# Autodesk Inventor assembly: PS20027
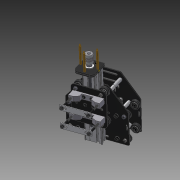
[picture p0: Inventor's stored thumbnail of the model, 180x180]
Saved by Autodesk Inventor 2014 (Build 180170000, 170)
## iProperties
Created: 2013-03-06
Part Number: PS20027
Document SubType Name: Assembly
Designer: Edward
Mass: 1567.3 g
Surface Area: 2632.04 cm^2
Volume: 388.503 cm^3
Density: 4.03421 g/cm^3
Author: Edward
## Documents named in this file (34)
- C:\Users\Edward\Documents\GitHub\Shapeoko_2\Autodesk_Inventor_Project\PS20027.iam
- C:\Users\Edward\Documents\GitHub\Shapeoko_2\Autodesk_Inventor_Project\25142-07.ipt
- C:\Users\Edward\Documents\GitHub\Shapeoko_2\Autodesk_Inventor_Project\25287-02.ipt
- C:\Users\Edward\Documents\GitHub\Shapeoko_2\Autodesk_Inventor_Project\25284-02.ipt
- C:\Users\Edward\Documents\GitHub\Shapeoko_2\Autodesk_Inventor_Project\25287-03.ipt
- C:\Users\Edward\Documents\GitHub\Shapeoko_2\Autodesk_Inventor_Project\PS20021.iam
- C:\Users\Edward\Documents\GitHub\Shapeoko_2\Autodesk_Inventor_Project\26016-01.ipt
- C:\Users\Edward\Documents\GitHub\Shapeoko_2\Autodesk_Inventor_Project\PS20002.ipt
- C:\Users\Edward\Documents\GitHub\Shapeoko_2\Autodesk_Inventor_Project\PS20005.ipt
- C:\Users\Edward\Documents\GitHub\Shapeoko_2\Autodesk_Inventor_Project\PS20014.ipt
- C:\Users\Edward\Documents\GitHub\Shapeoko_2\Autodesk_Inventor_Project\25286-01.ipt
- C:\Users\Edward\Documents\GitHub\Shapeoko_2\Autodesk_Inventor_Project\25772-02.ipt
- C:\Users\Edward\Documents\GitHub\Shapeoko_2\Autodesk_Inventor_Project\PS20011.ipt
- C:\Users\Edward\Documents\GitHub\Shapeoko_2\Autodesk_Inventor_Project\PS20007.ipt
- C:\Users\Edward\Documents\GitHub\Shapeoko_2\Autodesk_Inventor_Project\30288-01.ipt
- C:\Users\Edward\Documents\GitHub\Shapeoko_2\Autodesk_Inventor_Project\30169-01.ipt
- C:\Users\Edward\Documents\GitHub\Shapeoko_2\Autodesk_Inventor_Project\30289-01.ipt
- C:\Users\Edward\Documents\GitHub\Shapeoko_2\Autodesk_Inventor_Project\30287-01.ipt
- C:\Users\Edward\Documents\GitHub\Shapeoko_2\Autodesk_Inventor_Project\PS20015.ipt
- C:\Users\Edward\Documents\GitHub\Shapeoko_2\Autodesk_Inventor_Project\25286-02.ipt
- C:\Users\Edward\Documents\GitHub\Shapeoko_2\Autodesk_Inventor_Project\PS20010.ipt
- C:\Users\Edward\Documents\GitHub\Shapeoko_2\Autodesk_Inventor_Project\30158-01.ipt
- C:\Users\Edward\Documents\GitHub\Shapeoko_2\Autodesk_Inventor_Project\25203-02.iam
- C:\Users\Edward\Documents\GitHub\Shapeoko_2\Autodesk_Inventor_Project\25312-14.ipt
- C:\Users\Edward\Documents\GitHub\Shapeoko_2\Autodesk_Inventor_Project\25286-05.ipt
- C:\Users\Edward\Documents\GitHub\Shapeoko_2\Autodesk_Inventor_Project\PS20012.ipt
- C:\Users\Edward\Documents\GitHub\Shapeoko_2\Autodesk_Inventor_Project\PS20013.ipt
- C:\Users\Edward\Documents\GitHub\Shapeoko_2\Autodesk_Inventor_Project\25285-10.ipt
- C:\Users\Edward\Documents\GitHub\Shapeoko_2\Autodesk_Inventor_Project\PS20016.ipt
- C:\Users\Edward\Documents\GitHub\Shapeoko_2\Autodesk_Inventor_Project\PS20022.iam
- C:\Users\Edward\Documents\GitHub\Shapeoko_2\Autodesk_Inventor_Project\25312-20.ipt
- C:\Users\Edward\Documents\GitHub\Shapeoko_2\Autodesk_Inventor_Project\PS20006.ipt
- C:\Users\Edward\Documents\GitHub\Shapeoko_2\Autodesk_Inventor_Project\PS20004.ipt
- C:\Users\Edward\Documents\GitHub\Shapeoko_2\Autodesk_Inventor_Project\PS20017.ipt
## Components (147 placed, 34 different names)
1. 25142-07:1 — Mate:10, Flush:11, Flush:15, Mate:23, Mate:24, Flush:17, Insert:128, Insert:129, Angle:2, Mate:49, Flush:25
2. PS20021:1 [sub-assembly] — Mate:10, Flush:11, Flush:15, Flush:16, Insert:218, Insert:220, Insert:233, Insert:235, Insert:238, Insert:239, Insert:241, Insert:243, Insert:245, Insert:247, Insert:249, Insert:251
3. 25772-02:1
4. 30288-01:1 — Mate:25, Mate:26, Mate:28, Flush:17, Insert:115, Insert:116, Insert:117, Mate:32, Flush:18, Mate:47, Mate:48
5. 30288-01:2 — Insert:108, Mate:28, Insert:131, Insert:132, Insert:133
6. 30169-01:1 — Insert:108, Mate:25, Mate:26, Insert:109, Insert:110, Mate:53
7. PS20007:1 — Insert:109
8. PS20007:2 — Insert:110
9. 25287-03:2 — Insert:115, Insert:188
10. 25287-03:3 — Insert:116, Insert:187
11. 25287-03:4 — Insert:117, Insert:186
12. 30289-01:1 — Insert:128, Insert:129, Mate:32, Insert:136, Insert:137, Flush:18
13. PS20011:2 — Mate:33
14. 30287-01:1 — Insert:140, Insert:141, Insert:152, Angle:2, Mate:37, Insert:153, Insert:156, Insert:158, Insert:159, Insert:160, Insert:161, Insert:165, Insert:166, Mate:39, Insert:172, Mate:42, Insert:181, Insert:194, Insert:195, Mate:49, Flush:25
15. PSM3-01 — Insert:133, Insert:191
16. PS20015:4 — Insert:132, Insert:192
17. PS20015:5 — Insert:131, Insert:193
18. PS20004:9 — Insert:134
19. 25287-02:36 — Insert:134, Insert:136
20. PS20004:8 — Insert:135
21. 25287-02:37 — Insert:135, Insert:137
22. PS20010:1 — Insert:140, Insert:141, Mate:33
23. 30158-01:4 — Insert:152, Mate:38
24. 25287-02:45 — Insert:156, Insert:157
25. 25203-02:7 [sub-assembly] — Mate:37, Insert:154, Insert:155
26. 25284-02:13 — Insert:157
27. 25312-14:1 — Insert:153, Insert:154
28. 25286-05:1 — Insert:155
29. PS20012:1 — Insert:158, Insert:159, Insert:179, Mate:50, Flush:26, Flush:27, Insert:197
30. PS20012:2 — Insert:160, Insert:161, Mate:51, Flush:28, Flush:29, Mate:52
31. 25287-02:48 — Insert:166
32. 25203-02:8 [sub-assembly]
33. 25284-02:15
34. 25312-14:2 — Insert:165
35. 25286-05:2
36. 25203-02:9 [sub-assembly]
37. 25312-14:3 — Mate:38, Mate:39
38. 25286-05:3
39. 30158-01:5 — Insert:172, Mate:41
40. 25203-02:10 [sub-assembly]
41. 25312-14:4 — Mate:41, Mate:42
42. 25286-05:4
43. PS20016:1 — Mate:47, Insert:189
44. PS20016:2 — Mate:48, Insert:190
45. PS20014:9
46. PS20014:11
47. PS20014:12
48. 25285-10:1 — Insert:188
49. 25285-10:2 — Insert:187
50. 25285-10:3 — Insert:186
51. PS20016:3 — Insert:189
52. PS20016:4 — Insert:190
53. PS20015:6 — Insert:191
54. PS20015:7 — Insert:192
55. PS20015:8 — Insert:193
56. 25286-02:10 — Insert:194
57. 25286-02:11 — Insert:195
58. PS20013:3 — Mate:50, Flush:26, Flush:27, Mate:51
59. PS20013:4 — Flush:28, Flush:29, Mate:52
60. PS20022:1 [sub-assembly] — Insert:201, Insert:204, Insert:207, Insert:210, Insert:212, Insert:214, Insert:215, Insert:216, Insert:221, Insert:223, Insert:225, Insert:227, Insert:229, Insert:231, Insert:253
61. 25312-20:1 — Insert:219, Insert:220
62. PS20006:6 — Insert:217
63. PS20004:1 — Insert:199
64. 25203-02:12 [sub-assembly] — Insert:199, Insert:200
65. 25287-02:68 — Insert:200, Insert:201
66. 25284-02:23 — Insert:222
67. 25284-02:24 — Insert:211
68. 25287-02:71 — Insert:217, Insert:218
69. 25284-02:26 — Insert:213
70. 25287-02:72 — Insert:222, Insert:223
71. 25287-02:73 — Insert:213, Insert:214
72. 25287-02:74 — Insert:211, Insert:212
73. 30158-01:6 — Insert:215
74. 30158-01:7 — Insert:216
75. PS20004:5
76. 25203-02:15 [sub-assembly]
77. 25287-02:75 — Insert:204
78. PS20004:6
79. 25203-02:16 [sub-assembly]
80. 25287-02:76 — Insert:207
81. PS20004:7
82. 25203-02:17 [sub-assembly]
83. 25287-02:77 — Insert:210
84. PS20002:1 — Insert:219, Insert:221
85. 25284-02:30
86. 25287-02:78 — Insert:225
87. 25284-02:31
88. 25287-02:79 — Insert:227
89. 25284-02:32
90. 25287-02:80 — Insert:229
91. 25284-02:33
92. 25287-02:81 — Insert:231
93. PS20006:7
94. 25287-02:82 — Insert:233
95. PS20006:8
96. 25287-02:83 — Insert:235
97. PS20006:9
98. 25287-02:84 — Insert:239
99. PS20006:10
100. 25287-02:85 — Insert:238
101. 25312-20:7
102. PS20002:2 — Insert:241
103. 25312-20:8
104. PS20002:3 — Insert:243
105. 25312-20:9
106. PS20002:4 — Insert:245
107. 25312-20:10 — Insert:247
108. PS20002:5
109. PS20006:11
110. 25287-02:86 — Insert:249
111. 25312-20:11 — Insert:251
112. PS20002:6
113. 25284-02:34
114. 25287-02:87 — Insert:253
115. PS20017:1 — Mate:53
116. 26016-01:5 — Mate:23, Mate:24, Flush:16, Insert:104
117. 25287-02:35 — Insert:103, Insert:104
118. 25286-01:1 — Insert:103
119. 26016-01:6
120. 25287-02:53
121. 25286-01:2
122. 26016-01:7
123. 25287-02:54
124. 25286-01:3
125. 26016-01:8
126. 25287-02:55
127. 25286-01:4
128. 25286-02:3 — Insert:179
129. 25287-02:56 — Insert:181
130. 25284-02:16
131. 25286-02:7
132. 25287-02:57
133. 25284-02:17
134. 25286-02:8
135. 25287-02:58
136. 25284-02:18
137. 25286-02:9
138. 25287-02:59
139. 25284-02:19
140. PS20005:7
141. 25287-02:60 — Insert:197
142. PS20005:8
143. 25287-02:61
144. PS20005:9
145. 25287-02:62
146. PS20005:10
147. 25287-02:63
## Component patterns: (4 elements, first: 26016-01:5 + 25287-02:35 + 25286-01:1), (4 elements, first: 25286-02:3 + 25287-02:56 + 25284-02:16), (4 elements, first: PS20005:7 + 25287-02:60)
## Relationships (143: Insert 109, Mate 23, Flush 10, Angle 1)
- Mate:10: 25142-07:1 ↔ PS20021:1
- Flush:11 (-60 mm): 25142-07:1 ↔ PS20021:1
- Flush:15: 25142-07:1 ↔ PS20021:1
- Insert:103: 25287-02:35 ↔ 25286-01:1
- Mate:23: 25142-07:1 ↔ 26016-01:5
- Mate:24 (1 mm): 25142-07:1 ↔ 26016-01:5
- Flush:16 (2.5 mm): PS20021:1 ↔ 26016-01:5
- Insert:104 (5.4163 mm): 26016-01:5 ↔ 25287-02:35
- Insert:108 (0.5 mm): 30288-01:2 ↔ 30169-01:1
- Mate:25: 30288-01:1 ↔ 30169-01:1
- Mate:26: 30288-01:1 ↔ 30169-01:1
- Mate:28: 30288-01:1 ↔ 30288-01:2
- Flush:17 (-5 mm): 25142-07:1 ↔ 30288-01:1
- Insert:109: 30169-01:1 ↔ PS20007:1
- Insert:110: 30169-01:1 ↔ PS20007:2
- Insert:115: 30288-01:1 ↔ 25287-03:2
- Insert:116: 30288-01:1 ↔ 25287-03:3
- Insert:117: 30288-01:1 ↔ 25287-03:4
- Insert:128: 25142-07:1 ↔ 30289-01:1
- Insert:129: 25142-07:1 ↔ 30289-01:1
- Mate:32: 30288-01:1 ↔ 30289-01:1
- Insert:131: 30288-01:2 ↔ PS20015:5
- Insert:132: 30288-01:2 ↔ PS20015:4
- Insert:133: 30288-01:2 ↔ PSM3-01
- Insert:134: PS20004:9 ↔ 25287-02:36
- Insert:135: PS20004:8 ↔ 25287-02:37
- Insert:136 (6.8137 mm): 30289-01:1 ↔ 25287-02:36
- Insert:137 (6.8137 mm): 30289-01:1 ↔ 25287-02:37
- Insert:140: 30287-01:1 ↔ PS20010:1
- Insert:141: 30287-01:1 ↔ PS20010:1
- Mate:33: PS20011:2 ↔ PS20010:1
- Insert:152: 30287-01:1 ↔ 30158-01:4
- Angle:2 (0 deg): 25142-07:1 ↔ 30287-01:1
- Mate:37: 30287-01:1 ↔ 25203-02:7
- Insert:153: 30287-01:1 ↔ 25312-14:1
- Insert:154: 25203-02:7 ↔ 25312-14:1
- Insert:155: 25203-02:7 ↔ 25286-05:1
- Insert:156: 30287-01:1 ↔ 25287-02:45
- Insert:157: 25287-02:45 ↔ 25284-02:13
- Insert:158: 30287-01:1 ↔ PS20012:1
- Insert:159: 30287-01:1 ↔ PS20012:1
- Insert:160: 30287-01:1 ↔ PS20012:2
- Insert:161: 30287-01:1 ↔ PS20012:2
- [Insert]: 25203-02:8 ↔ 25312-14:2
- [Insert]: 25203-02:8 ↔ 25286-05:2
- [Insert]: 25287-02:48 ↔ 25284-02:15
- Insert:165: 30287-01:1 ↔ 25312-14:2
- Insert:166: 30287-01:1 ↔ 25287-02:48
- [Insert]: 25203-02:9 ↔ 25312-14:3
- [Insert]: 25203-02:9 ↔ 25286-05:3
- Mate:38: 30158-01:4 ↔ 25312-14:3
- Mate:39: 30287-01:1 ↔ 25312-14:3
- Flush:18 (0.598 mm): 30288-01:1 ↔ 30289-01:1
- [Insert]: 25203-02:10 ↔ 25312-14:4
- [Insert]: 25203-02:10 ↔ 25286-05:4
- [Mate]: 30158-01:5 ↔ 25312-14:4
- Insert:172: 30287-01:1 ↔ 30158-01:5
- Mate:41: 30158-01:5 ↔ 25312-14:4
- Mate:42: 30287-01:1 ↔ 25312-14:4
- Insert:179: PS20012:1 ↔ 25286-02:3
- [Insert]: 25287-02:56 ↔ 25284-02:16
- Insert:181: 30287-01:1 ↔ 25287-02:56
- Insert:186: 25287-03:4 ↔ 25285-10:3
- Insert:187: 25287-03:3 ↔ 25285-10:2
- Insert:188: 25287-03:2 ↔ 25285-10:1
- [Mate]: PS20004:8 ↔ PS20016:1
- [Mate]: PS20004:9 ↔ PS20016:2
- Mate:47: 30288-01:1 ↔ PS20016:1
- Mate:48: 30288-01:1 ↔ PS20016:2
- Insert:189: PS20016:1 ↔ PS20016:3
- Insert:190: PS20016:2 ↔ PS20016:4
- Insert:191: PSM3-01 ↔ PS20015:6
- Insert:192: PS20015:4 ↔ PS20015:7
- Insert:193: PS20015:5 ↔ PS20015:8
- Insert:194: 30287-01:1 ↔ 25286-02:10
- Insert:195: 30287-01:1 ↔ 25286-02:11
- Mate:49 (12.7 mm): 25142-07:1 ↔ 30287-01:1
- Flush:25 (-25 mm): 25142-07:1 ↔ 30287-01:1
- Mate:50 (40 mm): PS20012:1 ↔ PS20013:3
- Flush:26: PS20012:1 ↔ PS20013:3
- Flush:27: PS20012:1 ↔ PS20013:3
- Mate:51 (40 mm): PS20012:2 ↔ PS20013:3
- Flush:28: PS20012:2 ↔ PS20013:4
- Flush:29: PS20012:2 ↔ PS20013:4
- [Insert]: PS20005:7 ↔ 25287-02:60
- Insert:197 (42 mm): PS20012:1 ↔ 25287-02:60
- Mate:52 (40 mm): PS20012:2 ↔ PS20013:4
- Insert:199: PS20004:1 ↔ 25203-02:12
- Insert:200: 25203-02:12 ↔ 25287-02:68
- Insert:201: PS20022:1 ↔ 25287-02:68
- [Insert]: PS20004:5 ↔ 25203-02:15
- [Insert]: 25203-02:15 ↔ 25287-02:75
- Insert:204: PS20022:1 ↔ 25287-02:75
- [Insert]: PS20004:6 ↔ 25203-02:16
- [Insert]: 25203-02:16 ↔ 25287-02:76
- Insert:207: PS20022:1 ↔ 25287-02:76
- [Insert]: PS20004:7 ↔ 25203-02:17
- [Insert]: 25203-02:17 ↔ 25287-02:77
- Insert:210: PS20022:1 ↔ 25287-02:77
- Insert:211: 25284-02:24 ↔ 25287-02:74
- Insert:212: PS20022:1 ↔ 25287-02:74
- Insert:213: 25284-02:26 ↔ 25287-02:73
- Insert:214: PS20022:1 ↔ 25287-02:73
- Insert:215: PS20022:1 ↔ 30158-01:6
- Insert:216: PS20022:1 ↔ 30158-01:7
- Insert:217: PS20006:6 ↔ 25287-02:71
- Insert:218: PS20021:1 ↔ 25287-02:71
- Insert:219: 25312-20:1 ↔ PS20002:1
- Insert:220: PS20021:1 ↔ 25312-20:1
- Insert:221: PS20022:1 ↔ PS20002:1
- Insert:222: 25284-02:23 ↔ 25287-02:72
- Insert:223: PS20022:1 ↔ 25287-02:72
- [Insert]: 25284-02:30 ↔ 25287-02:78
- Insert:225: PS20022:1 ↔ 25287-02:78
- [Insert]: 25284-02:31 ↔ 25287-02:79
- Insert:227: PS20022:1 ↔ 25287-02:79
- [Insert]: 25284-02:32 ↔ 25287-02:80
- Insert:229: PS20022:1 ↔ 25287-02:80
- [Insert]: 25284-02:33 ↔ 25287-02:81
- Insert:231: PS20022:1 ↔ 25287-02:81
- [Insert]: PS20006:7 ↔ 25287-02:82
- Insert:233: PS20021:1 ↔ 25287-02:82
- [Insert]: PS20006:8 ↔ 25287-02:83
- Insert:235: PS20021:1 ↔ 25287-02:83
- [Insert]: PS20006:9 ↔ 25287-02:84
- [Insert]: PS20006:10 ↔ 25287-02:85
- Insert:238: PS20021:1 ↔ 25287-02:85
- Insert:239: PS20021:1 ↔ 25287-02:84
- [Insert]: 25312-20:7 ↔ PS20002:2
- Insert:241: PS20021:1 ↔ PS20002:2
- [Insert]: 25312-20:8 ↔ PS20002:3
- Insert:243: PS20021:1 ↔ PS20002:3
- [Insert]: 25312-20:9 ↔ PS20002:4
- Insert:245: PS20021:1 ↔ PS20002:4
- [Insert]: 25312-20:10 ↔ PS20002:5
- Insert:247: PS20021:1 ↔ 25312-20:10
- [Insert]: PS20006:11 ↔ 25287-02:86
- Insert:249: PS20021:1 ↔ 25287-02:86
- [Insert]: 25312-20:11 ↔ PS20002:6
- Insert:251: PS20021:1 ↔ 25312-20:11
- [Insert]: 25284-02:34 ↔ 25287-02:87
- Insert:253: PS20022:1 ↔ 25287-02:87
- Mate:53: 30169-01:1 ↔ PS20017:1
## Named parameters: d159_d104 = 0 mm, d101_d55_d51 = 0 mm, d212_d101_d55_d51 = 0 mm, d254_d246 = 0 mm, d255_d247 = 0 mm, d256_d249 = 0 mm, d259_d246 = 0 mm, d260_d247 = 0 mm, d267_d259_d246 = 0 mm, d268_d260_d247 = 0 mm, d269_d262 = 0 mm, d293_d249 = 0 mm, d331_d137 = 0 mm, d344_d341 = 0 mm, d345_d342 = 0 mm, d347_d341 = 0 mm, d348_d342 = 0 mm, d350_d341 = 0 mm, d351_d342 = 0 mm, d366_d364 = 0 mm, d368_d364 = 0 mm, d370_d364 = 0 mm, d372_d364 = 0 mm, d374_d359 = 0 mm, d376_d359 = 0 mm, d378_d359 = 0 mm, d379_d359 = 0 mm, d382_d361 = 0 mm, d384_d361 = 0 mm, d386_d361 = 0 mm, d388_d361 = 0 mm, d390_d379_d359 = 0 mm, d392_d388_d361 = 0 mm, d394_d372_d364 = 0 mm
